# Autodesk Inventor assembly: Battery
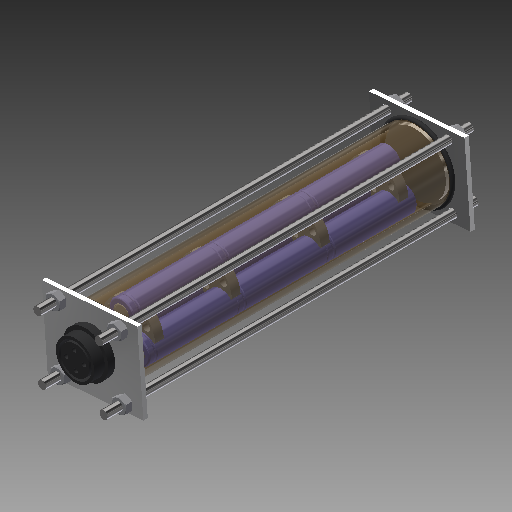
[picture p0: Inventor's stored thumbnail of the model, 512x512]
Saved by Autodesk Inventor 2018.1 (Build 221171000, 171)
## iProperties
Created: 2017-09-01
Part Number: Battery
Document SubType Name: Assembly
Designer: Kai
Author: Kai
## Documents named in this file (10)
- E:\robosub\Battery.iam
- E:\robosub\endcap1.ipt
- E:\robosub\polycarb_tube.ipt
- E:\robosub\gasket.ipt
- E:\robosub\18650.ipt
- E:\robosub\battery_holder.ipt
- E:\robosub\rod.ipt
- E:\robosub\endcap2.ipt
- E:\robosub\connector.ipt
- E:\robosub\6mm_nut.ipt
## Components (31 placed, 9 different names)
1. endcap1:1 — Mate:2, Mate:3, Mate:7, Mate:30, Mate:31, Mate:32, Mate:33, Mate:34, Flush:13, Flush:14, Flush:15, Mate:47, Mate:48, Mate:49, Mate:50
2. polycarb_tube:1 — Mate:2, Mate:3, Mate:4, Mate:6, Mate:29, Mate:35, Mate:36
3. gasket:1 — Mate:4, Mate:7
4. gasket:2 — Mate:6
5. 18650:1 — Mate:10, Flush:4, Mate:11, Flush:7, Mate:14, Mate:18
6. 18650:2 — Mate:9, Flush:5, Mate:12, Mate:13, Mate:17
7. 18650:3 — Mate:8, Flush:4, Flush:5, Flush:6, Mate:15, Mate:16, Mate:30
8. 18650:4 — Mate:15, Mate:16, Mate:23, Mate:24
9. 18650:5 — Mate:22, Mate:25
10. 18650:6 — Mate:23, Mate:24, Mate:28
11. 18650:7 — Mate:21, Mate:26, Flush:9, Mate:27
12. 18650:8 — Mate:14, Mate:18, Flush:8, Mate:20, Mate:21, Mate:26
13. 18650:9 — Mate:13, Mate:17, Mate:19, Mate:22, Mate:25
14. battery_holder:1 — Mate:11, Mate:12, Flush:7
15. battery_holder:2 — Mate:8, Mate:9, Mate:10, Flush:6, Mate:29
16. battery_holder:3 — Flush:8, Mate:19, Mate:20
17. battery_holder:4 — Flush:9, Mate:27, Mate:28
18. rod:1 — Mate:34, Flush:10, Mate:44, Mate:54
19. rod:2 — Mate:32, Flush:11, Mate:45, Mate:51
20. rod:3 — Mate:33, Flush:10, Flush:11, Flush:12, Flush:13, Mate:43, Mate:52
21. rod:4 — Mate:31, Flush:12, Mate:46, Mate:53
22. endcap2:1 — Mate:35, Mate:36, Flush:14, Flush:15, Mate:37, Mate:38, Mate:39, Mate:40, Mate:41, Mate:42
23. connector:1 — Mate:37, Mate:38
24. 6mm_nut:1 — Mate:41, Mate:43
25. 6mm_nut:2 — Mate:42, Mate:45
26. 6mm_nut:3 — Mate:40, Mate:46
27. 6mm_nut:4 — Mate:39, Mate:44
28. 6mm_nut:5 — Mate:47, Mate:51
29. 6mm_nut:6 — Mate:49, Mate:53
30. 6mm_nut:7 — Mate:48, Mate:52
31. 6mm_nut:8 — Mate:50, Mate:54
## Relationships (64: Mate 52, Flush 12)
- Mate:2: endcap1:1 ↔ polycarb_tube:1
- Mate:3: endcap1:1 ↔ polycarb_tube:1
- Mate:4: polycarb_tube:1 ↔ gasket:1
- Mate:6: polycarb_tube:1 ↔ gasket:2
- Mate:7: endcap1:1 ↔ gasket:1
- Mate:8: 18650:3 ↔ battery_holder:2
- Mate:9: 18650:2 ↔ battery_holder:2
- Mate:10: 18650:1 ↔ battery_holder:2
- Flush:4: 18650:1 ↔ 18650:3
- Flush:5: 18650:2 ↔ 18650:3
- Flush:6 (-5.08 mm): 18650:3 ↔ battery_holder:2
- Mate:11: 18650:1 ↔ battery_holder:1
- Mate:12: 18650:2 ↔ battery_holder:1
- Flush:7 (-3.81 mm): 18650:1 ↔ battery_holder:1
- Mate:13: 18650:2 ↔ 18650:9
- Mate:14: 18650:1 ↔ 18650:8
- Mate:15: 18650:3 ↔ 18650:4
- Mate:16: 18650:3 ↔ 18650:4
- Mate:17: 18650:2 ↔ 18650:9
- Mate:18: 18650:1 ↔ 18650:8
- Flush:8 (-3.81 mm): 18650:8 ↔ battery_holder:3
- Mate:19: 18650:9 ↔ battery_holder:3
- Mate:20: 18650:8 ↔ battery_holder:3
- Mate:21: 18650:7 ↔ 18650:8
- Mate:22: 18650:5 ↔ 18650:9
- Mate:23: 18650:4 ↔ 18650:6
- Mate:24: 18650:4 ↔ 18650:6
- Mate:25: 18650:5 ↔ 18650:9
- Mate:26: 18650:7 ↔ 18650:8
- Flush:9 (5.08 mm): 18650:7 ↔ battery_holder:4
- Mate:27: 18650:7 ↔ battery_holder:4
- Mate:28: 18650:6 ↔ battery_holder:4
- Mate:29: polycarb_tube:1 ↔ battery_holder:2
- Mate:30 (19.05 mm): endcap1:1 ↔ 18650:3
- Mate:31: endcap1:1 ↔ rod:4
- Mate:32: endcap1:1 ↔ rod:2
- Mate:33: endcap1:1 ↔ rod:3
- Mate:34: endcap1:1 ↔ rod:1
- Flush:10: rod:1 ↔ rod:3
- Flush:11: rod:2 ↔ rod:3
- Flush:12: rod:3 ↔ rod:4
- Flush:13 (-12.7 mm): endcap1:1 ↔ rod:3
- Mate:35: polycarb_tube:1 ↔ endcap2:1
- Mate:36: polycarb_tube:1 ↔ endcap2:1
- Flush:14: endcap1:1 ↔ endcap2:1
- Flush:15: endcap1:1 ↔ endcap2:1
- Mate:37: endcap2:1 ↔ connector:1
- Mate:38: endcap2:1 ↔ connector:1
- Mate:39: endcap2:1 ↔ 6mm_nut:4
- Mate:40: endcap2:1 ↔ 6mm_nut:3
- Mate:41: endcap2:1 ↔ 6mm_nut:1
- Mate:42: endcap2:1 ↔ 6mm_nut:2
- Mate:43: rod:3 ↔ 6mm_nut:1
- Mate:44: rod:1 ↔ 6mm_nut:4
- Mate:45: rod:2 ↔ 6mm_nut:2
- Mate:46: rod:4 ↔ 6mm_nut:3
- Mate:47: endcap1:1 ↔ 6mm_nut:5
- Mate:48: endcap1:1 ↔ 6mm_nut:7
- Mate:49: endcap1:1 ↔ 6mm_nut:6
- Mate:50: endcap1:1 ↔ 6mm_nut:8
- Mate:51: rod:2 ↔ 6mm_nut:5
- Mate:52: rod:3 ↔ 6mm_nut:7
- Mate:53: rod:4 ↔ 6mm_nut:6
- Mate:54: rod:1 ↔ 6mm_nut:8
